# Autodesk Inventor assembly: Microview_and_Headers
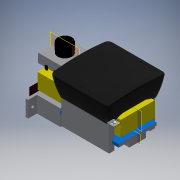
[picture p0: Inventor's stored thumbnail of the model, 180x180]
Saved by Autodesk Inventor 2019.4 (Build 234330000, 330)
## iProperties
Created: 2021-06-28
Part Number: Microview_and_Headers
Document SubType Name: Assembly
Designer: keshav
Author: keshav
## Documents named in this file (7)
- D:\Keshav\Maker\Microview_Pendant\Microview_Pendant\CAD\Microview_and_Headers.iam
- D:\Keshav\Micro Controlers\CAD of controllers\sparkfun-microview-oled-1.snapshot.3\Sparkfun display.ipt
- D:\Keshav\Maker\Microview_Pendant\Microview_Pendant\CAD\Female_Header_Spacer.ipt
- D:\Keshav\Maker\Microview_Pendant\Microview_Pendant\CAD\Wavgat_Battery_Charger.ipt
- D:\Keshav\Maker\Microview_Pendant\Microview_Pendant\CAD\Battery_37v_320mAh.ipt
- D:\Keshav\Maker\Microview_Pendant\Microview_Pendant\CAD\Push_Button.ipt
- D:\Keshav\Maker\Microview_Pendant\Microview_Pendant\CAD\Switch.ipt
## Components (7 placed, 6 different names)
1. Sparkfun display:1 — Flush:1, Flush:2, Mate:1
2. Female_Header_Spacer:1 — Flush:1, Flush:7
3. Female_Header_Spacer:2 — Flush:2, Flush:4, Flush:7
4. Wavgat_Battery_Charger:1 — Flush:3, Flush:4, Flush:6, Mate:6
5. Battery_37v_320mAh:1 — Mate:1, Flush:3, Mate:2, Mate:3, Mate:4
6. Push_Button:1 — Mate:2, Flush:5, Mate:4, Mate:5, Flush:8, Mate:6
7. Switch:1 — Flush:5, Mate:3, Mate:5, Flush:6, Flush:8
## Relationships (14: Flush 8, Mate 6)
- Flush:1 (1 mm): Sparkfun display:1 ↔ Female_Header_Spacer:1
- Flush:2 (1 mm): Sparkfun display:1 ↔ Female_Header_Spacer:2
- Mate:1: Sparkfun display:1 ↔ Battery_37v_320mAh:1
- Flush:3: Wavgat_Battery_Charger:1 ↔ Battery_37v_320mAh:1
- Flush:4 (3 mm): Female_Header_Spacer:2 ↔ Wavgat_Battery_Charger:1
- Mate:2 (2 mm): Battery_37v_320mAh:1 ↔ Push_Button:1
- Flush:5: Push_Button:1 ↔ Switch:1
- Mate:3 (2 mm): Battery_37v_320mAh:1 ↔ Switch:1
- Mate:4: Battery_37v_320mAh:1 ↔ Push_Button:1
- Mate:5: Push_Button:1 ↔ Switch:1
- Flush:6: Wavgat_Battery_Charger:1 ↔ Switch:1
- Flush:7: Female_Header_Spacer:1 ↔ Female_Header_Spacer:2
- Flush:8: Push_Button:1 ↔ Switch:1
- Mate:6: Wavgat_Battery_Charger:1 ↔ Push_Button:1
